# Autodesk Inventor assembly: Assembly1
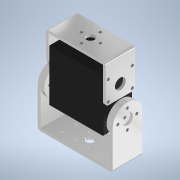
[picture p0: Inventor's stored thumbnail of the model, 180x180]
Saved by Autodesk Inventor 2021 (Build 250183000, 183)
## iProperties
Created: 2021-10-22
Part Number: Assembly1
Document SubType Name: Assembly
Designer: Asus
Author: Asus
## Documents named in this file (6)
- C:\Users\Asus\Desktop\Универстет\Третий Семестер\PD\Сборка Сервопривод.iam
- C:\Users\Asus\Desktop\Универстет\Третий Семестер\PD\Part1.ipt
- C:\Users\Asus\Desktop\Универстет\Третий Семестер\PD\Сервопривод.ipt
- C:\Users\Asus\Desktop\Универстет\Третий Семестер\PD\Part L.ipt
- C:\Users\Asus\Desktop\Универстет\Третий Семестер\PD\Part2.ipt
- C:\Users\Asus\Desktop\Универстет\Третий Семестер\PD\Part R.ipt
## Components (5 placed, 5 different names)
1. Part1:1 — Mate:1, Mate:3
2. Сервопривод:1 — Mate:1, Mate:2, Mate:3
3. Part L:1 — Mate:2, Mate:4
4. Part2:1 — Mate:4, Mate:5
5. Part R:1 — Mate:5
## Relationships (5: Mate 5)
- Mate:1: Part1:1 ↔ Сервопривод:1
- Mate:2: Сервопривод:1 ↔ Part L:1
- Mate:3: Part1:1 ↔ Сервопривод:1
- Mate:4: Part L:1 ↔ Part2:1
- Mate:5: Part2:1 ↔ Part R:1
